# Autodesk Inventor assembly: FK10 Fixed Side Support Unit
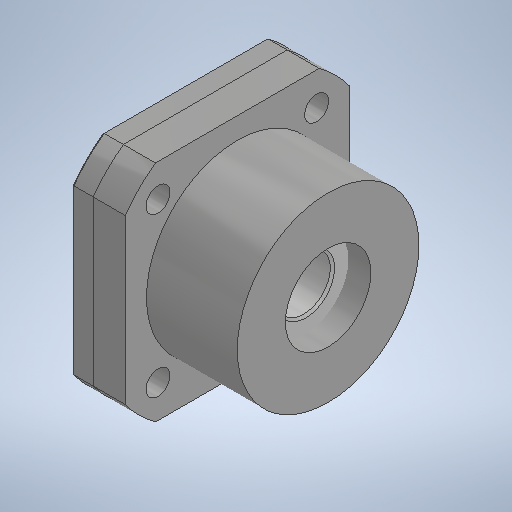
[picture p0: Inventor's stored thumbnail of the model, 512x512]
Saved by Autodesk Inventor 2025.2 (Build 292293000, 293)
## iProperties
Created: 2020-04-03
Part Number: FK10 Fixed Side Support Unit
Document SubType Name: Assembly
Designer: composite
Sending System: Autodesk Translation Framework v8.12.0.6
Preprocessor: ST-DEVELOPER v18
Title: C:/Users/gborozynski.POSTDATA/Downloads/sfu1204-ball-screw-450mm-500mm-900mm-1.snapshot.1 (1)/FK10 Fixed Side Support Unit.step
## Documents named in this file (4)
- H:\01-Members Space\Sam Munro\Extrusion Printer\Printer V2\FK10 Fixed Side Support Unit\FK10 Fixed Side Support Unit\FK10 Fixed Side Support Unit.iam
- H:\01-Members Space\Sam Munro\Extrusion Printer\Printer V2\FK10 Fixed Side Support Unit\FK10 Fixed Side Support Unit\5972K94.ipt
- H:\01-Members Space\Sam Munro\Extrusion Printer\Printer V2\FK10 Fixed Side Support Unit\FK10 Fixed Side Support Unit\92855A402.ipt
- H:\01-Members Space\Sam Munro\Extrusion Printer\Printer V2\FK10 Fixed Side Support Unit\FK10 Fixed Side Support Unit\Part17.ipt
## Components (7 placed, 3 different names)
1. 5972K94:1
2. 5972K94:2
3. 92855A402:1 — Flush:1
4. 92855A402:2 — Flush:2, Flush:3
5. 92855A402:3 — Flush:1, Flush:3
6. 92855A402:4 — Flush:4
7. Part17 — Flush:2, Flush:4
## Relationships (4: Flush 4)
- Flush:1: 92855A402:1 ↔ 92855A402:3
- Flush:2: 92855A402:2 ↔ Part17
- Flush:3: 92855A402:2 ↔ 92855A402:3
- Flush:4: 92855A402:4 ↔ Part17
